# Autodesk Inventor assembly: WormGearLock
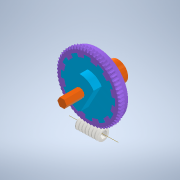
[picture p0: Inventor's stored thumbnail of the model, 180x180]
Saved by Autodesk Inventor 2021.2 (Build 252289000, 289)
## iProperties
Created: 2020-11-20
Part Number: WormGearLock
Document SubType Name: Assembly
Designer: robst
Author: robst
## Documents named in this file (6)
- C:\git\CAD-Development\robSteele\ShapeWays\TelescopeProjects\TelescopeMount\SplineLock\WormGearLock.iam
- C:\git\CAD-Development\robSteele\ShapeWays\TelescopeProjects\TelescopeMount\1_2x3-inchHexShaft.ipt
- C:\git\CAD-Development\robSteele\ShapeWays\TelescopeProjects\TelescopeMount\forkMountForDecTripV01\Design Accelerator\Worm Gears5.iam
- C:\git\CAD-Development\robSteele\ShapeWays\TelescopeProjects\TelescopeMount\1_2x1-hexBushing.ipt
- C:\git\CAD-Development\robSteele\ShapeWays\TelescopeProjects\TelescopeMount\SplineLock\gearLock.ipt
- C:\git\CAD-Development\robSteele\ShapeWays\TelescopeProjects\TelescopeMount\1_2x2x3_16-hexBearing.ipt
## Components (5 placed, 5 different names)
1. 1_2x3-inchHexShaft:1 — Mate:1, Mate:2, Mate:3
2. Worm Gears:1 [sub-assembly] — Insert:1, Flush:1
3. 1_2x1-hexBushing:1 — Insert:1, Insert:2, Mate:1, Mate:2, Mate:3
4. 1_2x2x3_16-hexBearing:1 — Insert:2, Insert:3
5. gearLock:1 — Insert:3, Flush:1
## Relationships (7: Insert 3, Mate 3, Flush 1)
- Insert:1: Worm Gears:1 ↔ 1_2x1-hexBushing:1
- Insert:2: 1_2x1-hexBushing:1 ↔ 1_2x2x3_16-hexBearing:1
- Insert:3: 1_2x2x3_16-hexBearing:1 ↔ gearLock:1
- Mate:1 (12.7 mm): 1_2x3-inchHexShaft:1 ↔ 1_2x1-hexBushing:1
- Mate:2: 1_2x3-inchHexShaft:1 ↔ 1_2x1-hexBushing:1
- Mate:3: 1_2x3-inchHexShaft:1 ↔ 1_2x1-hexBushing:1
- Flush:1: Worm Gears:1 ↔ gearLock:1
